# Autodesk Inventor assembly: WhitePumpStepperAdaptorV2
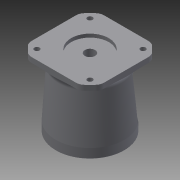
[picture p0: Inventor's stored thumbnail of the model, 180x180]
Saved by Autodesk Inventor 2013 (Build 170138000, 138)
## iProperties
Created: 2014-07-16
Part Number: WhitePumpStepperAdaptorV2
Document SubType Name: Assembly
Designer: Dan
Author: Dan
## Documents named in this file (3)
- H:\User Files\Fitzgerald\peristaltic pump\WhitePumpStepperAdaptor\WhitePumpStepperAdaptorV2.iam
- H:\User Files\Fitzgerald\peristaltic pump\WhitePumpStepperAdaptor\Parts\WhitePumpBase.ipt
- H:\User Files\Fitzgerald\peristaltic pump\WhitePumpStepperAdaptor\Parts\BearingHolderPlate.ipt
## Components (2 placed, 2 different names)
1. WhitePumpBase:1 — Flush:1
2. BearingHolderPlate:1 — Flush:1
## Relationships (1: Flush 1)
- Flush:1: WhitePumpBase:1 ↔ BearingHolderPlate:1
